# Autodesk Inventor assembly: cubi
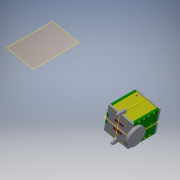
[picture p0: Inventor's stored thumbnail of the model, 180x180]
Saved by Autodesk Inventor 2019 (Build 230136000, 136)
## iProperties
Created: 2018-09-20
Part Number: cubi
Material: Générique
Document SubType Name: Assembly
Designer: Jérémy
Author: Jérémy
## Documents named in this file (9)
- D:\Utilisateurs\Jérémy\Documents\Programmation\cubi\mechanics\new_tiny\cubi.iam
- D:\Utilisateurs\Jérémy\Documents\Programmation\cubi\mechanics\new_tiny\moteur.ipt
- D:\Utilisateurs\Jérémy\Documents\Programmation\cubi\mechanics\new_tiny\box.ipt
- D:\Utilisateurs\Jérémy\Documents\Programmation\cubi\mechanics\new_tiny\board.ipt
- D:\Utilisateurs\Jérémy\Documents\Programmation\cubi\mechanics\new_tiny\bat9V.ipt
- D:\Utilisateurs\Jérémy\Documents\Programmation\cubi\mechanics\new_tiny\connector9V.ipt
- D:\Utilisateurs\Jérémy\Documents\Programmation\cubi\mechanics\new_tiny\support_card.ipt
- D:\Utilisateurs\Jérémy\Documents\Programmation\cubi\mechanics\new_tiny\small_wheel.ipt
- D:\Utilisateurs\Jérémy\Documents\Programmation\cubi\mechanics\new_tiny\cotes.xlsx
## Components (9 placed, 7 different names)
1. moteur:1 — Placage:1, Affleurement:1, Affleurement:2, Logement:3
2. moteur:2 — Placage:1, Affleurement:1, Affleurement:2, Affleurement:3, Affleurement:4, Affleurement:7
3. box:1 — Affleurement:3, Affleurement:4, Placage:2, Placage:3
4. board:1 — Logement:2, Affleurement:6
5. bat9V:1 — Logement:1, Affleurement:5
6. connector9V:1 — Logement:1, Affleurement:5, Logement:2
7. support_card:1 — Affleurement:6, Placage:2, Placage:3
8. small_wheel:1 — Affleurement:7
9. small_wheel:2 — Logement:3
## Relationships (13: Flush 7, Mate 3, Insert 3)
- Placage:1 [Mate] (25 mm): moteur:1 ↔ moteur:2
- Affleurement:1 [Flush]: moteur:1 ↔ moteur:2
- Affleurement:2 [Flush]: moteur:1 ↔ moteur:2
- Affleurement:3 [Flush]: moteur:2 ↔ box:1
- Affleurement:4 [Flush]: moteur:2 ↔ box:1
- Logement:1 [Insert]: bat9V:1 ↔ connector9V:1
- Affleurement:5 [Flush]: bat9V:1 ↔ connector9V:1
- Logement:2 [Insert]: board:1 ↔ connector9V:1
- Affleurement:6 [Flush]: board:1 ↔ support_card:1
- Placage:2 [Mate]: box:1 ↔ support_card:1
- Placage:3 [Mate]: box:1 ↔ support_card:1
- Affleurement:7 [Flush]: moteur:2 ↔ small_wheel:1
- Logement:3 [Insert]: moteur:1 ↔ small_wheel:2
## Named parameters: epaisseur = 6 mm, ecartement = 25 mm, dvis = 3 mm, largeur = 32 mm, L_fente = 30 mm, L_attache_carte = 15 mm, marge_attache_carte = 5 mm, marge_trou = 2 mm, taille_trou = 7 mm, L_moteur = 28.3 mm, largeur_cubi = 81.6 mm, L_cubi = 81.6 mm, H_cubi = 81.6 mm, epaisseur_wheel = 9 mm, d_wheel = 60 mm, H_nez = 25 mm, H_trou_nez = 10 mm, L_trou_int = 1 mm, chanfrein = 0.5 mm, H_trou_int = 0.2 mm, pos_trou_int_2 = 3 mm, pos_trou_int_1 = 0.7 mm, epaisseur_modules = 6 mm, L_modules = 20 mm, L_metabois = 8.2 mm, epaisseur_metabois = 3 mm
